# Autodesk Inventor assembly: Bicho
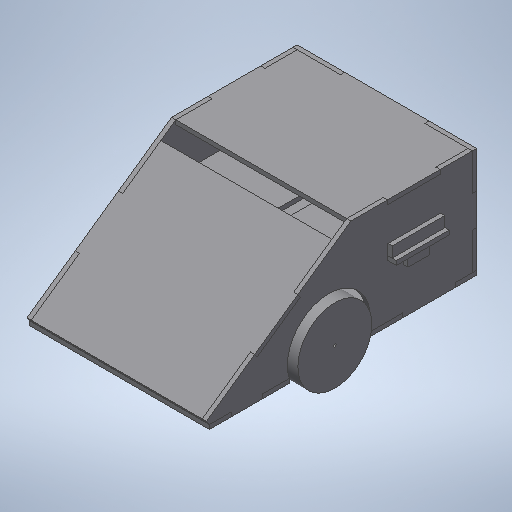
[picture p0: Inventor's stored thumbnail of the model, 512x512]
Saved by Autodesk Inventor 2025 (Build 290162000, 162)
## iProperties
Created: 2024-10-07
Part Number: Bicho
Document SubType Name: Assembly
Designer: feder
Author: feder
## Documents named in this file (13)
- C:\Users\feder\OneDrive - Universidad de Antioquia\Desktop\UdeA\2024-2\Electrónica\Bicho\Bicho.iam
- C:\Users\feder\OneDrive - Universidad de Antioquia\Desktop\UdeA\2024-2\Electrónica\Bicho\Parte inf.ipt
- C:\Users\feder\OneDrive - Universidad de Antioquia\Desktop\UdeA\2024-2\Electrónica\Bicho\Rueda Derecha.ipt
- C:\Users\feder\OneDrive - Universidad de Antioquia\Desktop\UdeA\2024-2\Electrónica\Bicho\Rueda Izquierda.ipt
- C:\Users\feder\OneDrive - Universidad de Antioquia\Desktop\UdeA\2024-2\Electrónica\Bicho\Bateria.ipt
- C:\Users\feder\OneDrive - Universidad de Antioquia\Desktop\UdeA\2024-2\Electrónica\Bicho\Puente H.ipt
- C:\Users\feder\OneDrive - Universidad de Antioquia\Desktop\UdeA\2024-2\Electrónica\Bicho\Rueda loca.ipt
- C:\Users\feder\OneDrive - Universidad de Antioquia\Desktop\UdeA\2024-2\Electrónica\Bicho\Tapa Tracera.ipt
- C:\Users\feder\OneDrive - Universidad de Antioquia\Desktop\UdeA\2024-2\Electrónica\Bicho\Tapa lateral 1.ipt
- C:\Users\feder\OneDrive - Universidad de Antioquia\Desktop\UdeA\2024-2\Electrónica\Bicho\Rampa.ipt
- C:\Users\feder\OneDrive - Universidad de Antioquia\Desktop\UdeA\2024-2\Electrónica\Bicho\Tapa Superior.ipt
- C:\Users\feder\OneDrive - Universidad de Antioquia\Desktop\UdeA\2024-2\Electrónica\Bicho\Parte intermedia.ipt
- C:\Users\feder\OneDrive - Universidad de Antioquia\Desktop\UdeA\2024-2\Electrónica\Bicho\Seguro.ipt
## Components (14 placed, 12 different names)
1. Parte inf:1 — Mate:1, Mate:2, Flush:1, Flush:2, Mate:4, Flush:3, Flush:4, Mate:5, Flush:5, Mate:6, Flush:7, Mate:7, Flush:9
2. Rueda Izquierda:1 — Mate:1, Flush:2, Mate:3
3. Rueda Derecha:1 — Mate:2, Flush:1, Mate:3
4. Tapa Tracera:1 — Mate:4, Flush:3, Flush:4, Flush:6, Flush:8, Mate:9, Mate:10, Flush:12, Mate:11, Mate:14
5. Tapa lateral 1:1 — Mate:5, Flush:5, Flush:6, Flush:10, Mate:12, Mate:18
6. Tapa lateral 1:2 — Mate:6, Flush:7, Flush:8, Flush:11, Mate:8, Mate:15
7. Rueda loca:1 — Mate:7, Flush:9
8. Rampa:1 — Flush:10, Flush:11, Mate:8
9. Tapa Superior:1 — Mate:9, Mate:10, Flush:12
10. Puente H:1
11. Parte intermedia:1 — Mate:11, Mate:12, Mate:13, Mate:14, Mate:16, Mate:17, Mate:19, Mate:20
12. Bateria:1 — Mate:13
13. Seguro:1 — Mate:15, Mate:16, Mate:17
14. Seguro:2 — Mate:18, Mate:19, Mate:20
## Relationships (32: Mate 20, Flush 12)
- Mate:1: Parte inf:1 ↔ Rueda Izquierda:1
- Mate:2: Parte inf:1 ↔ Rueda Derecha:1
- Flush:1: Parte inf:1 ↔ Rueda Derecha:1
- Flush:2: Parte inf:1 ↔ Rueda Izquierda:1
- Mate:3: Rueda Izquierda:1 ↔ Rueda Derecha:1
- Mate:4: Parte inf:1 ↔ Tapa Tracera:1
- Flush:3: Parte inf:1 ↔ Tapa Tracera:1
- Flush:4: Parte inf:1 ↔ Tapa Tracera:1
- Mate:5: Parte inf:1 ↔ Tapa lateral 1:1
- Flush:5: Parte inf:1 ↔ Tapa lateral 1:1
- Flush:6: Tapa Tracera:1 ↔ Tapa lateral 1:1
- Mate:6: Parte inf:1 ↔ Tapa lateral 1:2
- Flush:7: Parte inf:1 ↔ Tapa lateral 1:2
- Flush:8: Tapa Tracera:1 ↔ Tapa lateral 1:2
- Mate:7: Parte inf:1 ↔ Rueda loca:1
- Flush:9 (15 mm): Parte inf:1 ↔ Rueda loca:1
- Flush:10: Tapa lateral 1:1 ↔ Rampa:1
- Flush:11: Tapa lateral 1:2 ↔ Rampa:1
- Mate:8: Tapa lateral 1:2 ↔ Rampa:1
- Mate:9: Tapa Tracera:1 ↔ Tapa Superior:1
- Mate:10: Tapa Tracera:1 ↔ Tapa Superior:1
- Flush:12: Tapa Tracera:1 ↔ Tapa Superior:1
- Mate:11: Tapa Tracera:1 ↔ Parte intermedia:1
- Mate:12: Tapa lateral 1:1 ↔ Parte intermedia:1
- Mate:13: Parte intermedia:1 ↔ Bateria:1
- Mate:14: Tapa Tracera:1 ↔ Parte intermedia:1
- Mate:15: Tapa lateral 1:2 ↔ Seguro:1
- Mate:16: Parte intermedia:1 ↔ Seguro:1
- Mate:17: Parte intermedia:1 ↔ Seguro:1
- Mate:18: Tapa lateral 1:1 ↔ Seguro:2
- Mate:19: Parte intermedia:1 ↔ Seguro:2
- Mate:20: Parte intermedia:1 ↔ Seguro:2
